# Autodesk Inventor assembly: Field_Assy
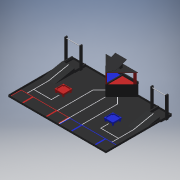
[picture p0: Inventor's stored thumbnail of the model, 180x180]
Saved by Autodesk Inventor 2017 (Build 210142000, 142)
## iProperties
Created: 2017-04-14
Part Number: Field_Assy
Document SubType Name: Assembly
Designer: Alex Tacescu
Author: Alex Tacescu
## Documents named in this file (6)
- C:\Users\alext\Documents\School\WPI\Spring 2017\RBE 1001\Final Project\Field Parts\Field_Assy.iam
- C:\Users\alext\Documents\School\WPI\Spring 2017\RBE 1001\Final Project\Field Parts\Field.ipt
- C:\Users\alext\Documents\School\WPI\Spring 2017\RBE 1001\Final Project\Field Parts\Barn and Rad.ipt
- C:\Users\alext\Documents\School\WPI\Spring 2017\RBE 1001\Final Project\Field Parts\Perch.ipt
- C:\Users\alext\Documents\School\WPI\Spring 2017\RBE 1001\Final Project\Field Parts\Ramp.ipt
- C:\Users\alext\Documents\School\WPI\Spring 2017\RBE 1001\Final Project\Field Parts\Pen.ipt
## Components (8 placed, 5 different names)
1. Field:1 — Flush:1, Flush:2, Flush:3, Mate:1, Mate:2, Mate:3, Mate:4, Mate:5, Mate:6, Mate:7, Mate:8, Mate:9, Mate:11, Mate:12, Mate:13, Mate:15, Mate:16
2. Barn and Rad:1 — Mate:1, Mate:2, Flush:4
3. Perch:1 — Mate:3, Mate:4, Mate:5, Mate:14
4. Perch:2 — Mate:6, Mate:7, Mate:8, Mate:10
5. Ramp:1 — Mate:9, Mate:10, Mate:11
6. Ramp:2 — Mate:12, Mate:13, Mate:14
7. Pen:1 — Mate:15
8. Pen:2 — Mate:16
## Relationships (20: Mate 16, Flush 4)
- Flush:1: Field:1
- Flush:2: Field:1
- Flush:3: Field:1
- Mate:1: Field:1 ↔ Barn and Rad:1
- Mate:2: Field:1 ↔ Barn and Rad:1
- Flush:4: Barn and Rad:1
- Mate:3: Field:1 ↔ Perch:1
- Mate:4: Field:1 ↔ Perch:1
- Mate:5: Field:1 ↔ Perch:1
- Mate:6: Field:1 ↔ Perch:2
- Mate:7: Field:1 ↔ Perch:2
- Mate:8: Field:1 ↔ Perch:2
- Mate:9: Field:1 ↔ Ramp:1
- Mate:10: Perch:2 ↔ Ramp:1
- Mate:11: Field:1 ↔ Ramp:1
- Mate:12: Field:1 ↔ Ramp:2
- Mate:13: Field:1 ↔ Ramp:2
- Mate:14: Perch:1 ↔ Ramp:2
- Mate:15: Field:1 ↔ Pen:1
- Mate:16: Field:1 ↔ Pen:2
